# Autodesk Inventor assembly: Base
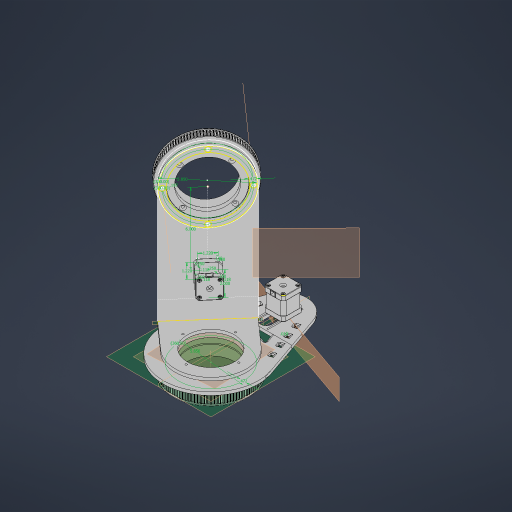
[picture p0: Inventor's stored thumbnail of the model, 512x512]
Saved by Autodesk Inventor 2024 (Build 280153000, 153)
## iProperties
Created: 2023-10-21
Part Number: Base
Document SubType Name: Assembly
Designer: range
Author: range
## Documents named in this file (7)
- C:\Users\range\CodingProjects\C-AAM\CAD\V1\Base.iam
- C:\Users\range\CodingProjects\C-AAM\CAD\V1\Parts\LazySusan.iam
- C:\Users\range\CodingProjects\C-AAM\CAD\V1\LargePitchAssembly.iam
- C:\Users\range\CodingProjects\C-AAM\CAD\V1\WCP-0562\WCP-0562.ipt
- C:\Users\range\CodingProjects\C-AAM\CAD\V1\6627T91_Stepper Motor\6627T91_Stepper Motor.ipt
- C:\Users\range\CodingProjects\C-AAM\CAD\V1\Parts\2ndAxis.iam
- C:\Users\range\CodingProjects\C-AAM\CAD\V1\BoardAssembly.iam
## Components (6 placed, 6 different names)
1. LazySusan:1 [sub-assembly] — Mate:7, Flush:4, Mate:12, Mate:13
2. LargePitchAssembly:1 [sub-assembly] — Mate:7, Flush:5
3. WCP-0562:1 — Mate:5, Angle:2, Flush:5, Mate:20
4. 6627T91_Stepper Motor:1 — Mate:5, Angle:2
5. 2ndAxis:1 [sub-assembly] — Flush:4, Mate:12, Mate:13, Mate:16
6. BoardAssembly:1 [sub-assembly]
## Relationships (23: Mate 16, Flush 5, Angle 2)
- [Mate] (2.5 mm): LazySusan:1 ↔ LargePitchAssembly:1
- [Mate]: LazySusan:1 ↔ LargePitchAssembly:1
- [Flush]: LazySusan:1 ↔ BoardAssembly:1
- [Flush]: LazySusan:1 ↔ BoardAssembly:1
- [Mate]: 6627T91_Stepper Motor:1 ↔ BoardAssembly:1
- Mate:5: WCP-0562:1 ↔ 6627T91_Stepper Motor:1
- [Mate]: LazySusan:1 ↔ BoardAssembly:1
- Mate:7: LazySusan:1 ↔ LargePitchAssembly:1
- [Mate]: LazySusan:1 ↔ BoardAssembly:1
- [Mate]: LazySusan:1 ↔ BoardAssembly:1
- Flush:4: LazySusan:1 ↔ 2ndAxis:1
- Mate:12: LazySusan:1 ↔ 2ndAxis:1
- Mate:13: LazySusan:1 ↔ 2ndAxis:1
- [Angle] (0 deg): 6627T91_Stepper Motor:1 ↔ BoardAssembly:1
- [Mate]: 6627T91_Stepper Motor:1 ↔ BoardAssembly:1
- Angle:2 (180 deg): WCP-0562:1 ↔ 6627T91_Stepper Motor:1
- Flush:5: LargePitchAssembly:1 ↔ WCP-0562:1
- Mate:16: 2ndAxis:1
- Mate:17
- [Mate]: BoardAssembly:1
- [Mate]: BoardAssembly:1
- Mate:20: WCP-0562:1
- [Flush]: BoardAssembly:1
